# Autodesk Inventor assembly: Assembly1.0
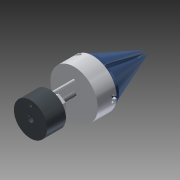
[picture p0: Inventor's stored thumbnail of the model, 180x180]
Saved by Autodesk Inventor 2015 (Build 190159000, 159)
## iProperties
Created: 2016-04-14
Part Number: Assembly1.0
Document SubType Name: Assembly
Designer: Diogo Figueiredo
Author: Diogo Figueiredo
## Documents named in this file (6)
- C:\Users\Diogo Figueiredo\Desktop\App\Assembly1.0.iam
- C:\Users\Diogo Figueiredo\Desktop\App\Body.ipt
- C:\Users\Diogo Figueiredo\Desktop\App\Pá 120.ipt
- C:\Users\Diogo Figueiredo\Desktop\App\Nut.ipt
- C:\Users\Diogo Figueiredo\Desktop\App\Bearing.ipt
- C:\Users\Diogo Figueiredo\Desktop\App\Engine.ipt
## Components (7 placed, 5 different names)
1. Body:1 — Mate:3, Mate:4, Mate:5
2. Pá 120:1
3. Pá 120:2
4. Pá 120:3
5. Nut:1 — Mate:3, Mate:6
6. Bearing:1 — Mate:1, Mate:2, Mate:4, Mate:6
7. Engine:1 — Mate:1, Mate:2, Mate:5
## Relationships (6: Mate 6)
- Mate:1: Bearing:1 ↔ Engine:1
- Mate:2: Bearing:1 ↔ Engine:1
- Mate:3: Body:1 ↔ Nut:1
- Mate:4: Body:1 ↔ Bearing:1
- Mate:5: Body:1 ↔ Engine:1
- Mate:6: Nut:1 ↔ Bearing:1
